# Autodesk Inventor assembly: Piston Guide Holder assy
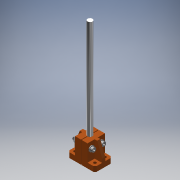
[picture p0: Inventor's stored thumbnail of the model, 180x180]
Saved by Autodesk Inventor 2018 (Build 220112000, 112)
## iProperties
Created: 2017-09-27
Part Number: Piston Guide Holder assy
Document SubType Name: Assembly
Designer: Gabriel Smolnycki
Author: Gabriel Smolnycki
## Documents named in this file (6)
- H:\dev\planb\mechanics\V1INV\Subassemblies\Piston Guide Holder assy.iam
- H:\dev\planb\mechanics\V1INV\Piston\Piston Guide Holder.ipt
- H:\dev\planb\mechanics\V1INV\Piston\Piston Guide Rod 8mm.ipt
- H:\dev\planb\mechanics\V1INV\Hardware\M4x30 SS SHCS.ipt
- H:\dev\planb\mechanics\V1INV\Hardware\M4 SS Washer.ipt
- H:\dev\planb\mechanics\V1INV\Hardware\M4 SS Locknut.ipt
## Components (11 placed, 5 different names)
1. Piston Guide Holder:1 — Insert:1, Mate:1, Insert:5, Insert:6
2. Piston Guide Holder:2 — Insert:2, Mate:1, Insert:3, Insert:4
3. Piston Guide Rod 8mm:1 — Insert:1, Insert:2
4. M4x30 SS SHCS:1 — Insert:8
5. M4x30 SS SHCS:2 — Insert:7
6. M4 SS Washer:1 — Insert:3, Insert:7
7. M4 SS Washer:2 — Insert:4, Insert:8
8. M4 SS Washer:3 — Insert:6, Insert:9
9. M4 SS Washer:5 — Insert:5, Insert:10
10. M4 SS Locknut:1 — Insert:10
11. M4 SS Locknut:2 — Insert:9
## Relationships (11: Insert 10, Mate 1)
- Insert:1: Piston Guide Holder:1 ↔ Piston Guide Rod 8mm:1
- Insert:2: Piston Guide Holder:2 ↔ Piston Guide Rod 8mm:1
- Mate:1: Piston Guide Holder:1 ↔ Piston Guide Holder:2
- Insert:3: Piston Guide Holder:2 ↔ M4 SS Washer:1
- Insert:4: Piston Guide Holder:2 ↔ M4 SS Washer:2
- Insert:5: Piston Guide Holder:1 ↔ M4 SS Washer:5
- Insert:6: Piston Guide Holder:1 ↔ M4 SS Washer:3
- Insert:7: M4x30 SS SHCS:2 ↔ M4 SS Washer:1
- Insert:8: M4x30 SS SHCS:1 ↔ M4 SS Washer:2
- Insert:9: M4 SS Washer:3 ↔ M4 SS Locknut:2
- Insert:10: M4 SS Washer:5 ↔ M4 SS Locknut:1
